# Autodesk Inventor assembly: AR-100
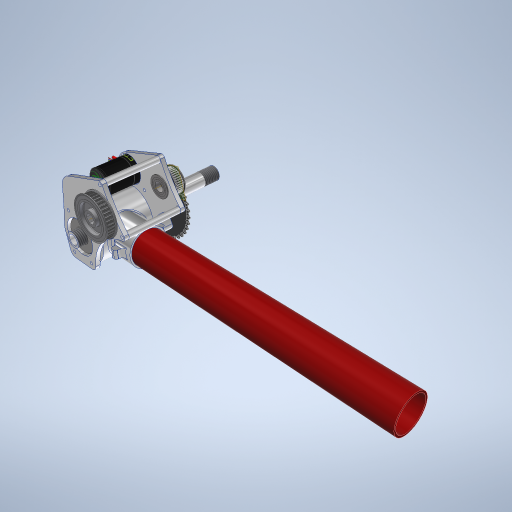
[picture p0: Inventor's stored thumbnail of the model, 512x512]
Saved by Autodesk Inventor 2023.4 (Build 274418000, 418)
## iProperties
Created: 2025-01-22
Part Number: AR-100
Document SubType Name: Assembly
Designer: slick
Author: slick
## Documents named in this file (15)
- C:\Users\mavericks\Documents\Robotics\GitHub\2025-ReefScape---CAD\Arm\AR-100.iam
- C:\Users\mavericks\Documents\Robotics\GitHub\2025-ReefScape---CAD\Arm\AR-001.ipt
- C:\Users\mavericks\Documents\Robotics\GitHub\2025-ReefScape---CAD\Arm\AR-002.ipt
- C:\Users\mavericks\Documents\Robotics\GitHub\2025-ReefScape---CAD\COMMON PARTS\BEARINGS\0_875_ID_x_1_875_OD_X_0_500_Radial_Bearing_EE11S-2RS.ipt
- C:\Users\mavericks\Documents\Robotics\GitHub\2025-ReefScape---CAD\COMMON PARTS\MOTORS\Minion.ipt
- C:\Users\mavericks\Documents\Robotics\GitHub\2025-ReefScape---CAD\COMMON PARTS\BEARINGS\13_75mm_1_2_ThunderHex_ID_x_1_125_OD_x_0_313_WD_Flanged_Bearing_217-4006_MIR.ipt
- C:\Users\mavericks\Documents\Robotics\GitHub\2025-ReefScape---CAD\COMMON PARTS\PULLEYS\gt2\16T Gt2 Kracken PullyWCP-1178.ipt
- C:\Users\mavericks\Documents\Robotics\GitHub\2025-ReefScape---CAD\COMMON PARTS\PULLEYS\gt2\36t_x_9mm_Wide_Double_Flange_Aluminum_Pulley_GT2_3mm_1_2_Hex_Bore_217-5873.ipt
- C:\Users\mavericks\Documents\Robotics\GitHub\2025-ReefScape---CAD\COMMON PARTS\PULLEYS\htd\36t_x_9mm_Wide_Double_Flange_Aluminum_Pulley_HTD_5mm_1_2_Hex_Bore_217-3231.ipt
- C:\Users\mavericks\Documents\Robotics\GitHub\2025-ReefScape---CAD\Arm\AR-003.ipt
- C:\Users\mavericks\Documents\Robotics\GitHub\2025-ReefScape---CAD\Arm\AR-005.ipt
- C:\Users\mavericks\Documents\Robotics\GitHub\2025-ReefScape---CAD\Arm\AR-006.ipt
- C:\Users\mavericks\Documents\Robotics\GitHub\2025-ReefScape---CAD\Arm\AR-007.ipt
- C:\Users\mavericks\Documents\Robotics\GitHub\2025-ReefScape---CAD\COMMON PARTS\SPROCKETS\35\WCP-0983\WCP-0983.ipt
- C:\Users\mavericks\Documents\Robotics\GitHub\2025-ReefScape---CAD\Arm\AR-009.ipt
## Components (17 placed, 14 different names)
1. AR-001:1 — Mate:1, Mate:2, Mate:3, Mate:4, Insert:1, Insert:2, Mate:13, Mate:14, Insert:17, Insert:18
2. AR-002:1 — Insert:1, Insert:2, Mate:5, Insert:4, Mate:8, Insert:5, Insert:19, Insert:20
3. 0_875_ID_x_1_875_OD_X_0_500_Radial_Bearing_EE11S-2RS:1 — Mate:1, Mate:3, Mate:15, Flush:2
4. 0_875_ID_x_1_875_OD_X_0_500_Radial_Bearing_EE11S-2RS:2 — Mate:2, Mate:4
5. Minion:1 — Mate:5, Mate:7, Flush:1, Mate:8, Insert:5
6. 13_75mm_1_2_ThunderHex_ID_x_1_125_OD_x_0_313_WD_Flanged_Bearing_217-4006_MIR:1 — Insert:4, Mate:9
7. 16T Gt2 Kracken PullyWCP-1178:1 — Mate:7, Flush:1, Mate:10
8. 36t_x_9mm_Wide_Double_Flange_Aluminum_Pulley_GT2_3mm_1_2_Hex_Bore_217-5873:1 — Mate:9, Mate:10, Mate:11
9. 36t_x_9mm_Wide_Double_Flange_Aluminum_Pulley_HTD_5mm_1_2_Hex_Bore_217-3231:1 — Mate:11, Mate:16
10. 13_75mm_1_2_ThunderHex_ID_x_1_125_OD_x_0_313_WD_Flanged_Bearing_217-4006_MIR:2 — Insert:14, Mate:16
11. AR-005:1 — Mate:13, Mate:14
12. AR-006:1 — Mate:15, Flush:2
13. AR-007:1 — Insert:14, Insert:15, Insert:16, Insert:17, Insert:18
14. AR-003:1 — Insert:16
15. AR-003:2 — Insert:15
16. WCP-0983:1 — Insert:21, Insert:22, Insert:23, Insert:24
17. AR-009:1 — Insert:19, Insert:20, Insert:21, Insert:22, Insert:23, Insert:24
## Relationships (31: Insert 15, Mate 14, Flush 2)
- Mate:1: AR-001:1 ↔ 0_875_ID_x_1_875_OD_X_0_500_Radial_Bearing_EE11S-2RS:1
- Mate:2: AR-001:1 ↔ 0_875_ID_x_1_875_OD_X_0_500_Radial_Bearing_EE11S-2RS:2
- Mate:3: AR-001:1 ↔ 0_875_ID_x_1_875_OD_X_0_500_Radial_Bearing_EE11S-2RS:1
- Mate:4: AR-001:1 ↔ 0_875_ID_x_1_875_OD_X_0_500_Radial_Bearing_EE11S-2RS:2
- Insert:1: AR-001:1 ↔ AR-002:1
- Insert:2: AR-001:1 ↔ AR-002:1
- Mate:5: AR-002:1 ↔ Minion:1
- Insert:4: AR-002:1 ↔ 13_75mm_1_2_ThunderHex_ID_x_1_125_OD_x_0_313_WD_Flanged_Bearing_217-4006_MIR:1
- Mate:7: Minion:1 ↔ 16T Gt2 Kracken PullyWCP-1178:1
- Flush:1: Minion:1 ↔ 16T Gt2 Kracken PullyWCP-1178:1
- Mate:8: AR-002:1 ↔ Minion:1
- Insert:5: AR-002:1 ↔ Minion:1
- Mate:9: 13_75mm_1_2_ThunderHex_ID_x_1_125_OD_x_0_313_WD_Flanged_Bearing_217-4006_MIR:1 ↔ 36t_x_9mm_Wide_Double_Flange_Aluminum_Pulley_GT2_3mm_1_2_Hex_Bore_217-5873:1
- Mate:10: 16T Gt2 Kracken PullyWCP-1178:1 ↔ 36t_x_9mm_Wide_Double_Flange_Aluminum_Pulley_GT2_3mm_1_2_Hex_Bore_217-5873:1
- Mate:11: 36t_x_9mm_Wide_Double_Flange_Aluminum_Pulley_GT2_3mm_1_2_Hex_Bore_217-5873:1 ↔ 36t_x_9mm_Wide_Double_Flange_Aluminum_Pulley_HTD_5mm_1_2_Hex_Bore_217-3231:1
- Mate:13: AR-001:1 ↔ AR-005:1
- Mate:14 (-50.8 mm): AR-001:1 ↔ AR-005:1
- Mate:15: 0_875_ID_x_1_875_OD_X_0_500_Radial_Bearing_EE11S-2RS:1 ↔ AR-006:1
- Flush:2 (-12.7 mm): 0_875_ID_x_1_875_OD_X_0_500_Radial_Bearing_EE11S-2RS:1 ↔ AR-006:1
- Insert:14: 13_75mm_1_2_ThunderHex_ID_x_1_125_OD_x_0_313_WD_Flanged_Bearing_217-4006_MIR:2 ↔ AR-007:1
- Insert:15: AR-007:1 ↔ AR-003:2
- Insert:16: AR-007:1 ↔ AR-003:1
- Mate:16 (3.175 mm): 36t_x_9mm_Wide_Double_Flange_Aluminum_Pulley_HTD_5mm_1_2_Hex_Bore_217-3231:1 ↔ 13_75mm_1_2_ThunderHex_ID_x_1_125_OD_x_0_313_WD_Flanged_Bearing_217-4006_MIR:2
- Insert:17: AR-001:1 ↔ AR-007:1
- Insert:18: AR-001:1 ↔ AR-007:1
- Insert:19: AR-002:1 ↔ AR-009:1
- Insert:20: AR-002:1 ↔ AR-009:1
- Insert:21: WCP-0983:1 ↔ AR-009:1
- Insert:22: WCP-0983:1 ↔ AR-009:1
- Insert:23: WCP-0983:1 ↔ AR-009:1
- Insert:24: WCP-0983:1 ↔ AR-009:1
